# Autodesk Inventor assembly: caixa principal
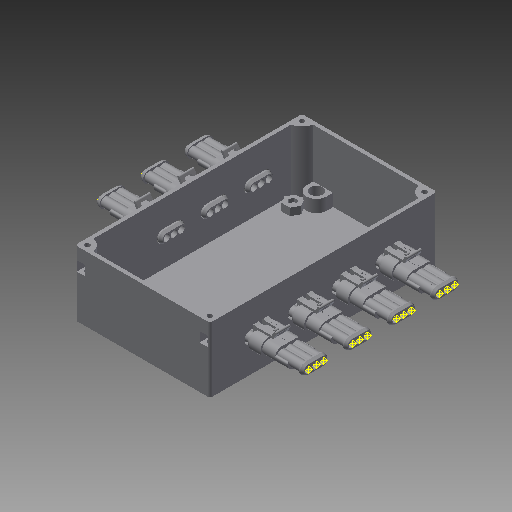
[picture p0: Inventor's stored thumbnail of the model, 512x512]
Saved by Autodesk Inventor 2019 (Build 230136000, 136)
## iProperties
Created: 2020-06-01
Part Number: caixa principal
Document SubType Name: Assembly
Designer: luiza
Author: luiza
## Documents named in this file (4)
- G:\Meu Drive\Projetos\Projeto 2020 2021\Eletrônica 2020-2021\Projeção mecânica\Caixas\Caixa Principal\caixa principal.iam
- G:\Meu Drive\Projetos\Projeto 2020 2021\Eletrônica 2020-2021\Projeção mecânica\Caixas\Caixa Principal\Base caixa principal.ipt
- G:\Meu Drive\Projetos\Projeto 2020 2021\Eletrônica 2020-2021\Projeção mecânica\Caixas\Caixa Principal\Tampa caixa principal.ipt
- G:\Meu Drive\Projetos\Projeto 2020 2021\Eletrônica 2020-2021\Projeção mecânica\Caixas\Caixa Principal\AMP 3 position.ipt
## Components (9 placed, 3 different names)
1. Base caixa principal:1 — Flush:1, Mate:1, Mate:2, Mate:3, Mate:4, Mate:5, Mate:6, Mate:7, Mate:8, Mate:9, Mate:10, Mate:11, Mate:12, Mate:13, Mate:14, Mate:15, Mate:16, Mate:17, Mate:18, Mate:19, Mate:20, Mate:21
2. Tampa caixa principal:1 — Flush:1
3. AMP 3 position:1 — Mate:1, Mate:2, Mate:3
4. AMP 3 position:2 — Mate:7, Mate:8, Mate:11
5. AMP 3 position:3 — Mate:9, Mate:10, Mate:12
6. AMP 3 position:4 — Mate:4, Mate:5, Mate:6
7. AMP 3 position:5 — Mate:17, Mate:18, Mate:21
8. AMP 3 position:6 — Mate:15, Mate:16, Mate:20
9. AMP 3 position:7 — Mate:13, Mate:14, Mate:19
## Relationships (22: Mate 21, Flush 1)
- Flush:1: Base caixa principal:1 ↔ Tampa caixa principal:1
- Mate:1: Base caixa principal:1 ↔ AMP 3 position:1
- Mate:2: Base caixa principal:1 ↔ AMP 3 position:1
- Mate:3: Base caixa principal:1 ↔ AMP 3 position:1
- Mate:4: Base caixa principal:1 ↔ AMP 3 position:4
- Mate:5: Base caixa principal:1 ↔ AMP 3 position:4
- Mate:6: Base caixa principal:1 ↔ AMP 3 position:4
- Mate:7: Base caixa principal:1 ↔ AMP 3 position:2
- Mate:8: Base caixa principal:1 ↔ AMP 3 position:2
- Mate:9: Base caixa principal:1 ↔ AMP 3 position:3
- Mate:10: Base caixa principal:1 ↔ AMP 3 position:3
- Mate:11: Base caixa principal:1 ↔ AMP 3 position:2
- Mate:12: Base caixa principal:1 ↔ AMP 3 position:3
- Mate:13: Base caixa principal:1 ↔ AMP 3 position:7
- Mate:14: Base caixa principal:1 ↔ AMP 3 position:7
- Mate:15: Base caixa principal:1 ↔ AMP 3 position:6
- Mate:16: Base caixa principal:1 ↔ AMP 3 position:6
- Mate:17: Base caixa principal:1 ↔ AMP 3 position:5
- Mate:18: Base caixa principal:1 ↔ AMP 3 position:5
- Mate:19: Base caixa principal:1 ↔ AMP 3 position:7
- Mate:20: Base caixa principal:1 ↔ AMP 3 position:6
- Mate:21: Base caixa principal:1 ↔ AMP 3 position:5
